# Autodesk Inventor assembly: 1m_E2C_10_06_018_0___E2_100_06_12PZ_A1_1
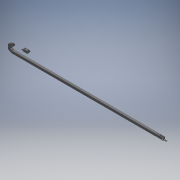
[picture p0: Inventor's stored thumbnail of the model, 180x180]
Saved by Autodesk Inventor 2019.3 (Build 233278000, 278)
## iProperties
Company: CADClick - www.CADClick.com
Created: 2020-08-23
Part Number: 1m_E2C_10_06_018_0___E2_100_06_12PZ_A1_1
Material: Generisch
Description: STEP AP214
Document SubType Name: Assembly
Designer: Nicolas Frick
Authority: unknown authorization
Preprocessor: Spatial InterOp 3D
Title: cctmp_6B86B663-61F8-438B-AAAD-12B288EE78A7_2020_08_24_01_55_25_0565..stp
Author: igus GmbH
Revision Number: NONE
## Documents named in this file (8)
- C:\Users\Nicolas Frick\Sync\OneDrive\airhockeybot\mechanical_design\inventor\igus\1m_E2C_10_06_018_0___E2_100_06_12PZ_A1_1.iam
- C:\Users\Nicolas Frick\Sync\OneDrive\airhockeybot\mechanical_design\inventor\igus\2020_08_24_01_55_25_0549.ipt
- C:\Users\Nicolas Frick\Sync\OneDrive\airhockeybot\mechanical_design\inventor\igus\2020_08_24_01_55_25_0518.ipt
- C:\Users\Nicolas Frick\Sync\OneDrive\airhockeybot\mechanical_design\inventor\igus\2020_08_24_01_55_25_0487.ipt
- C:\Users\Nicolas Frick\Sync\OneDrive\airhockeybot\mechanical_design\inventor\igus\2020_08_24_01_55_25_0456.ipt
- C:\Users\Nicolas Frick\Sync\OneDrive\airhockeybot\mechanical_design\inventor\igus\2020_08_24_01_55_25_0424.ipt
- C:\Users\Nicolas Frick\Sync\OneDrive\airhockeybot\mechanical_design\inventor\igus\2020_08_24_01_55_25_0393.ipt
- C:\Users\Nicolas Frick\Sync\OneDrive\airhockeybot\mechanical_design\inventor\igus\2020_08_24_01_55_25_0362.ipt
## Components (7 placed, 7 different names)
1. 2020_08_24_01_55_25_0549
2. 2020_08_24_01_55_25_0518 — Drehbar:1
3. 2020_08_24_01_55_25_0487
4. 2020_08_24_01_55_25_0456
5. 2020_08_24_01_55_25_0424
6. 2020_08_24_01_55_25_0393 — Drehbar:1
7. 2020_08_24_01_55_25_0362
## Relationships (1: RevoluteJoint 1)
- Drehbar:1 [RevoluteJoint]: 2020_08_24_01_55_25_0518 ↔ 2020_08_24_01_55_25_0393
